# Autodesk Inventor assembly: Housing_Assembly_V3
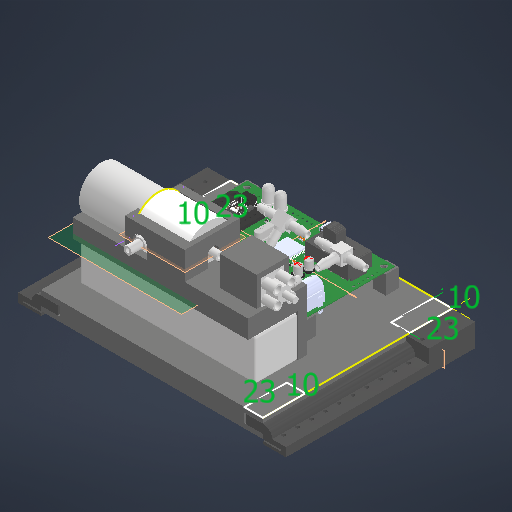
[picture p0: Inventor's stored thumbnail of the model, 512x512]
Saved by Autodesk Inventor 2026.2 (Build 302298000, 298)
## iProperties
Created: 2026-03-09
Part Number: Housing_Assembly_V3
Document SubType Name: Assembly
Designer: vckot
Author: vckot
## Documents named in this file (13)
- C:\Users\vckot\OneDrive\Documents\Vaibhav\capstone\CAD_files\Version_3\Housing_Assembly_V3.iam
- C:\Users\vckot\OneDrive\Documents\Vaibhav\capstone\CAD_files\PCB_Housing\TourniquetPCBV1_Updated\TourniquetPCBV1_Updated\TourniquetPCBV1_Updated.iam
- C:\Users\vckot\OneDrive\Documents\Vaibhav\capstone\CAD_files\Batteries\Battery_Small.ipt
- C:\Users\vckot\OneDrive\Documents\Vaibhav\capstone\CAD_files\PCB_Housing\PCB_Housing_01_V3.ipt
- C:\Users\vckot\OneDrive\Documents\Vaibhav\capstone\CAD_files\Motor_Valve\Adafruit_1528-4663-ND.ipt
- C:\Users\vckot\OneDrive\Documents\Vaibhav\capstone\CAD_files\Motor\Adafruit_1528_4699_ND.ipt
- C:\Users\vckot\OneDrive\Documents\Vaibhav\capstone\CAD_files\Pipe_Connectors\Adafruit_4662.ipt
- C:\Users\vckot\OneDrive\Documents\Vaibhav\capstone\CAD_files\PCB_Housing\PCB_Housing_02_V3.ipt
- C:\Users\vckot\OneDrive\Documents\Vaibhav\capstone\CAD_files\PCB_Housing\PCB_Housing_03_V3.ipt
- C:\Users\vckot\OneDrive\Documents\Vaibhav\capstone\CAD_files\PCB_Housing\PCB_Housing_04_V3.ipt
- C:\Users\vckot\OneDrive\Documents\Vaibhav\capstone\CAD_files\PCB_Housing\PCB_Housing_05_V3.ipt
- C:\Users\vckot\OneDrive\Documents\Vaibhav\capstone\CAD_files\Snap_Switch\Snap_Switch_Assembly.iam
- C:\Users\vckot\OneDrive\Documents\Vaibhav\capstone\CAD_files\Tourniquet_Rails\Tourniquet_Rail_01_V3.ipt
## Components (13 placed, 12 different names)
1. Snap_Switch_Assembly:1 [sub-assembly] — Mate:20, Flush:22, Flush:15
2. TourniquetPCBV1_Updated:1 [sub-assembly] — Flush:1, Flush:2, Flush:3, Mate:1, Flush:4, Mate:2, Mate:3, Mate:4
3. Battery_Small:1 — Mate:1, Flush:4, Mate:14, Flush:6, Flush:7, Mate:8, Angle:6, Mate:16, Flush:8
4. PCB_Housing_01_V3:1 — Mate:2, Mate:3, Mate:4, Mate:14, Mate:15, Mate:19, Flush:13, Flush:14, Mate:21, Flush:23, Flush:24
5. Adafruit_1528-4663-ND:1 — Mate:5, Mate:6, Mate:9, Mate:11, Angle:4, Angle:6, Flush:11, Flush:12
6. Adafruit_1528_4699_ND:1 — Angle:1, Angle:2, Mate:5, Flush:6, Flush:7, Mate:6, Mate:8, Flush:10
7. Adafruit_4662:1 — Mate:9, Angle:4, Mate:11, Mate:12, Angle:7, Mate:13
8. Adafruit_4662:2 — Mate:12, Angle:7, Mate:13
9. PCB_Housing_02_V3:1 — Mate:15, Mate:16, Flush:8, Flush:9, Mate:17, Mate:18
10. PCB_Housing_03_V3:1 — Flush:9, Mate:17, Flush:10
11. PCB_Housing_04_V3:1 — Mate:18, Flush:11, Flush:12
12. PCB_Housing_05_V3:1 — Mate:19, Flush:13, Flush:14, Mate:20, Flush:22, Flush:15
13. Tourniquet_Rail_01_V3:1 — Mate:21, Flush:23, Flush:24
## Relationships (41: Mate 19, Flush 17, Angle 5)
- Flush:1: TourniquetPCBV1_Updated:1
- Flush:2: TourniquetPCBV1_Updated:1
- Flush:3: TourniquetPCBV1_Updated:1
- Mate:1 (10 mm): TourniquetPCBV1_Updated:1 ↔ Battery_Small:1
- Flush:4: TourniquetPCBV1_Updated:1 ↔ Battery_Small:1
- Mate:2: TourniquetPCBV1_Updated:1 ↔ PCB_Housing_01_V3:1
- Mate:3: TourniquetPCBV1_Updated:1 ↔ PCB_Housing_01_V3:1
- Mate:4: TourniquetPCBV1_Updated:1 ↔ PCB_Housing_01_V3:1
- Mate:14: Battery_Small:1 ↔ PCB_Housing_01_V3:1
- Angle:1 (180 deg): Adafruit_1528_4699_ND:1
- Angle:2 (0 deg): Adafruit_1528_4699_ND:1
- Mate:5: Adafruit_1528-4663-ND:1 ↔ Adafruit_1528_4699_ND:1
- Flush:6: Battery_Small:1 ↔ Adafruit_1528_4699_ND:1
- Flush:7: Battery_Small:1 ↔ Adafruit_1528_4699_ND:1
- Mate:6 (5 mm): Adafruit_1528-4663-ND:1 ↔ Adafruit_1528_4699_ND:1
- Mate:8 (3.5 mm): Battery_Small:1 ↔ Adafruit_1528_4699_ND:1
- Mate:9: Adafruit_1528-4663-ND:1 ↔ Adafruit_4662:1
- Angle:4 (0 deg): Adafruit_1528-4663-ND:1 ↔ Adafruit_4662:1
- Mate:11 (10 mm): Adafruit_1528-4663-ND:1 ↔ Adafruit_4662:1
- Angle:6 (0 deg): Battery_Small:1 ↔ Adafruit_1528-4663-ND:1
- Mate:12: Adafruit_4662:1 ↔ Adafruit_4662:2
- Angle:7 (-45 deg): Adafruit_4662:1 ↔ Adafruit_4662:2
- Mate:13 (5 mm): Adafruit_4662:1 ↔ Adafruit_4662:2
- Mate:15: PCB_Housing_01_V3:1 ↔ PCB_Housing_02_V3:1
- Mate:16: Battery_Small:1 ↔ PCB_Housing_02_V3:1
- Flush:8: Battery_Small:1 ↔ PCB_Housing_02_V3:1
- Flush:9: PCB_Housing_02_V3:1 ↔ PCB_Housing_03_V3:1
- Mate:17: PCB_Housing_02_V3:1 ↔ PCB_Housing_03_V3:1
- Flush:10 (-2.5 mm): Adafruit_1528_4699_ND:1 ↔ PCB_Housing_03_V3:1
- Mate:18: PCB_Housing_02_V3:1 ↔ PCB_Housing_04_V3:1
- Flush:11: Adafruit_1528-4663-ND:1 ↔ PCB_Housing_04_V3:1
- Flush:12 (-2.5 mm): Adafruit_1528-4663-ND:1 ↔ PCB_Housing_04_V3:1
- Mate:19: PCB_Housing_01_V3:1 ↔ PCB_Housing_05_V3:1
- Flush:13: PCB_Housing_01_V3:1 ↔ PCB_Housing_05_V3:1
- Flush:14: PCB_Housing_01_V3:1 ↔ PCB_Housing_05_V3:1
- Mate:20: Snap_Switch_Assembly:1 ↔ PCB_Housing_05_V3:1
- Flush:22: Snap_Switch_Assembly:1 ↔ PCB_Housing_05_V3:1
- Flush:15: Snap_Switch_Assembly:1 ↔ PCB_Housing_05_V3:1
- Mate:21: PCB_Housing_01_V3:1 ↔ Tourniquet_Rail_01_V3:1
- Flush:23: PCB_Housing_01_V3:1 ↔ Tourniquet_Rail_01_V3:1
- Flush:24: PCB_Housing_01_V3:1 ↔ Tourniquet_Rail_01_V3:1
